# Autodesk Inventor assembly: Motherboard_assembly
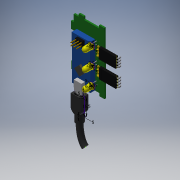
[picture p0: Inventor's stored thumbnail of the model, 180x180]
Saved by Autodesk Inventor 2016 (Build 200138000, 138)
## iProperties
Created: 2015-06-12
Part Number: Motherboard_assembly
Document SubType Name: Assembly
Designer: Openlab
Author: Openlab
## Documents named in this file (5)
- D:\Alexey\HS-Spectrophotometer\parts\Paris\Microcontroller_board_assumbly.iam
- D:\Alexey\HS-Spectrophotometer\parts\Paris\Microcontroller_board.ipt
- D:\Alexey\HS-Spectrophotometer\parts\Common\Pin-connector-angled-4.iam
- D:\Alexey\HS-Spectrophotometer\parts\Common\LED.ipt
- D:\Alexey\HS-Spectrophotometer\parts\Common\Mini_USB_cable.ipt
## Components (7 placed, 4 different names)
1. Microcontroller_board:1 — Mate:9, Mate:11, Mate:13, Mate:16, Mate:17, Mate:18, Mate:19, Mate:20, Mate:21, Mate:22, Mate:23, Mate:24, Mate:25, Mate:26, Mate:27
2. Pin-connector-angled-4:1 [sub-assembly] — Mate:19, Mate:20, Mate:21
3. Pin-connector-angled-4:2 [sub-assembly] — Mate:16, Mate:17, Mate:18
4. LED:1 — Mate:9, Mate:22
5. LED:2 — Mate:13, Mate:24
6. LED:3 — Mate:11, Mate:23
7. Mini_USB_cable:1 — Mate:25, Mate:26, Mate:27
## Relationships (15: Mate 15)
- Mate:9: Microcontroller_board:1 ↔ LED:1
- Mate:11: Microcontroller_board:1 ↔ LED:3
- Mate:13: Microcontroller_board:1 ↔ LED:2
- Mate:16: Microcontroller_board:1 ↔ Pin-connector-angled-4:2
- Mate:17: Microcontroller_board:1 ↔ Pin-connector-angled-4:2
- Mate:18: Microcontroller_board:1 ↔ Pin-connector-angled-4:2
- Mate:19: Microcontroller_board:1 ↔ Pin-connector-angled-4:1
- Mate:20: Microcontroller_board:1 ↔ Pin-connector-angled-4:1
- Mate:21: Microcontroller_board:1 ↔ Pin-connector-angled-4:1
- Mate:22 (8 mm): Microcontroller_board:1 ↔ LED:1
- Mate:23 (8 mm): Microcontroller_board:1 ↔ LED:3
- Mate:24 (8 mm): Microcontroller_board:1 ↔ LED:2
- Mate:25: Microcontroller_board:1 ↔ Mini_USB_cable:1
- Mate:26: Microcontroller_board:1 ↔ Mini_USB_cable:1
- Mate:27: Microcontroller_board:1 ↔ Mini_USB_cable:1
